# Autodesk Inventor assembly: echec2
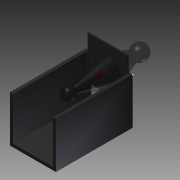
[picture p0: Inventor's stored thumbnail of the model, 180x180]
Saved by Autodesk Inventor 2015 (Build 190159000, 159)
## iProperties
Created: 2015-02-16
Part Number: echec2
Document SubType Name: Assembly
Designer: informatique
Author: informatique
## Documents named in this file (6)
- C:\Users\informatique\Documents\Mourey\echec2.iam
- C:\Users\informatique\Documents\Mourey\Pièce carré-01.ipt
- C:\Users\informatique\Documents\Mourey\socle.ipt
- C:\Users\informatique\Documents\Mourey\pion.ipt
- C:\Users\informatique\Documents\Mourey\Croisillon.ipt
- C:\Users\informatique\Documents\Mourey\fou.ipt
## Components (5 placed, 5 different names)
1. Pièce carré-01:1 — Placage:1, Placage:2, Placage:3
2. socle:1 — Placage:1, Placage:2, Placage:3, Placage:4, Placage:5, Placage:6, Placage:8, Placage:9
3. pion:1 — Placage:4, Placage:5, Placage:6, Placage:7
4. Croisillon:1 — Placage:7, Placage:8, Placage:9, Placage:10, Placage:11, Placage:12
5. fou:1 — Placage:10, Placage:11, Placage:12
## Relationships (12: Mate 12)
- Placage:1 [Mate]: Pièce carré-01:1 ↔ socle:1
- Placage:2 [Mate]: Pièce carré-01:1 ↔ socle:1
- Placage:3 [Mate]: Pièce carré-01:1 ↔ socle:1
- Placage:4 [Mate]: socle:1 ↔ pion:1
- Placage:5 [Mate]: socle:1 ↔ pion:1
- Placage:6 [Mate]: socle:1 ↔ pion:1
- Placage:7 [Mate]: pion:1 ↔ Croisillon:1
- Placage:8 [Mate]: socle:1 ↔ Croisillon:1
- Placage:9 [Mate]: socle:1 ↔ Croisillon:1
- Placage:10 [Mate]: Croisillon:1 ↔ fou:1
- Placage:11 [Mate]: Croisillon:1 ↔ fou:1
- Placage:12 [Mate]: Croisillon:1 ↔ fou:1
